# Autodesk Inventor assembly: Sprocket Axle and Wheel
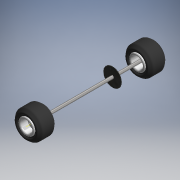
[picture p0: Inventor's stored thumbnail of the model, 180x180]
Saved by Autodesk Inventor 2016 (Build 200138000, 138)
## iProperties
Created: 2011-11-16
Part Number: Sprocket Axle and Wheel
Document SubType Name: Assembly
Designer: Matthew Cheung
Mass: 26663 g
Surface Area: 11661.8 cm^2
Volume: 17467.3 cm^3
Density: 1.52645 g/cm^3
Sending System: SolidWorks 2011
Last Author: Dennis Lieu
Last Saved: 2011-11-24
Author: Matthew Cheung
## Documents named in this file (5)
- C:\Users\jonathan\Desktop\CLEAN COPIES\GoCart Transmission\Inventor\Sprocket Axle and Wheel.iam
- C:\Users\jonathan\Desktop\CLEAN COPIES\GoCart Transmission\Inventor\Axle.ipt
- C:\Users\jonathan\Desktop\CLEAN COPIES\GoCart Transmission\Inventor\Rear Hub.ipt
- C:\Users\jonathan\Desktop\CLEAN COPIES\GoCart Transmission\Inventor\Rear Wheel.ipt
- C:\Users\jonathan\Desktop\CLEAN COPIES\GoCart Transmission\Inventor\driven sprocket - 6236K277.ipt
## Components (6 placed, 4 different names)
1. 0.5 axle:1 — Mate:1, Flush:1, Flush:2, Mate:8
2. rear_hub:1 — Mate:2, Mate:6, Flush:1
3. rear_hub:2 — Mate:4, Mate:7, Flush:2
4. rear_wheel:1 — Mate:3, Mate:6
5. rear_wheel:2 — Mate:5, Mate:7
6. driven sprocket - 6236K277:1 — Mate:8, Mate:9
## Relationships (11: Mate 9, Flush 2)
- Mate:1: 0.5 axle:1
- Mate:2: rear_hub:1
- Mate:3: rear_wheel:1
- Mate:4: rear_hub:2
- Mate:5: rear_wheel:2
- Mate:6: rear_hub:1 ↔ rear_wheel:1
- Flush:1: 0.5 axle:1 ↔ rear_hub:1
- Mate:7: rear_hub:2 ↔ rear_wheel:2
- Flush:2: 0.5 axle:1 ↔ rear_hub:2
- Mate:8: 0.5 axle:1 ↔ driven sprocket - 6236K277:1
- Mate:9: driven sprocket - 6236K277:1
